# Autodesk Inventor assembly: wheelhub
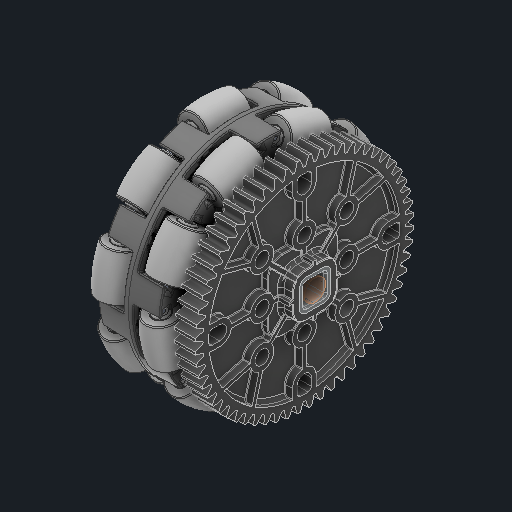
[picture p0: Inventor's stored thumbnail of the model, 512x512]
Saved by Autodesk Inventor 2025 (Build 290162000, 162)
## iProperties
Created: 2024-06-25
Part Number: wheelhub
Document SubType Name: Assembly
Designer: Audrey
Author: Audrey
## Documents named in this file (4)
- D:\vex_robotics_high_stakes\hardware\cad\EARLY_SEASON\chassis\drivebay\wheelhub.iam
- D:\vex_robotics_high_stakes\hardware\cad\VEX-CAD-Inventor\Motion\Wheels\Omni Wheel\2.75 Omni AS, No Insert.iam
- C:\Users\Audrey\vex_robotics_high_stakes\hardware\cad\VEX-CAD-Inventor\Motion\Wheels\Omni Wheel.iam
- D:\vex_robotics_high_stakes\hardware\cad\custom_parts\modified_parts\Half Cut HS 60T Gear.ipt
## Components (2 placed, 2 different names)
1. 2.75 Omni AS, No Insert:1 [sub-assembly] — Insert:1
2. Half Cut HS 60T Gear:1 — Insert:1
## Relationships (1: Insert 1)
- Insert:1 (3.9688 mm): 2.75 Omni AS, No Insert:1 ↔ Half Cut HS 60T Gear:1
